# Autodesk Inventor assembly: Assemblage
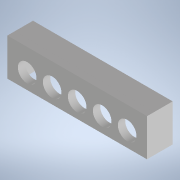
[picture p0: Inventor's stored thumbnail of the model, 180x180]
Saved by Autodesk Inventor 2020 (Build 240168000, 168)
## iProperties
Created: 2019-11-07
Part Number: Assemblage
Document SubType Name: Assembly
Designer: erwan
Author: erwan
## Documents named in this file (4)
- C:\Users\erwan\Desktop\Eirbot\Coupe robotique\Table\Ecueils\Assemblage.iam
- C:\Users\erwan\Desktop\Eirbot\Coupe robotique\Table\Ecueils\Support.ipt
- C:\Users\erwan\Desktop\Eirbot\Coupe robotique\Table\Ecueils\Fond.ipt
- C:\Users\erwan\Desktop\Eirbot\Coupe robotique\Table\Ecueils\Coté.ipt
## Components (4 placed, 3 different names)
1. Support:1 — Placage:1, Placage:2, Placage:3, Affleurement:1, Placage:4, Placage:7
2. Fond:1 — Placage:3, Affleurement:1, Placage:5, Placage:6, Placage:8, Placage:9
3. Coté:1 — Placage:7, Placage:8, Placage:9
4. Coté:2 — Placage:4, Placage:5, Placage:6
## Relationships (10: Mate 9, Flush 1)
- Placage:1 [Mate]: Support:1
- Placage:2 [Mate]: Support:1
- Placage:3 [Mate]: Support:1 ↔ Fond:1
- Affleurement:1 [Flush]: Support:1 ↔ Fond:1
- Placage:4 [Mate]: Support:1 ↔ Coté:2
- Placage:5 [Mate]: Fond:1 ↔ Coté:2
- Placage:6 [Mate]: Fond:1 ↔ Coté:2
- Placage:7 [Mate]: Support:1 ↔ Coté:1
- Placage:8 [Mate]: Fond:1 ↔ Coté:1
- Placage:9 [Mate]: Fond:1 ↔ Coté:1
